# Autodesk Inventor assembly: robotic_guitar
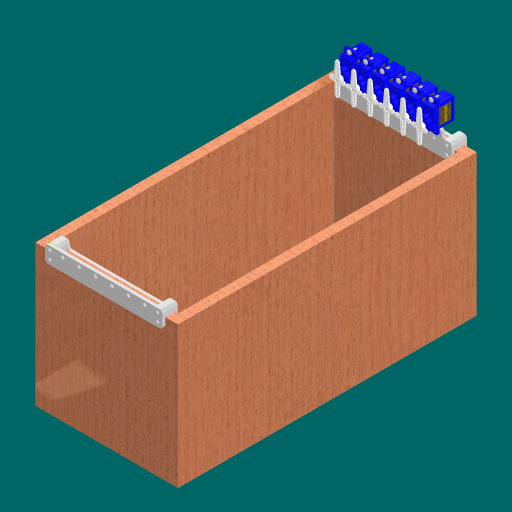
[picture p0: Inventor's stored thumbnail of the model, 512x512]
Saved by Autodesk Inventor 2023 (Build 270158000, 158)
## iProperties
Created: 2022-11-12
Part Number: robotic_guitar
Document SubType Name: Assembly
Designer: sgodi
Author: sgodi
## Documents named in this file (6)
- C:\Users\sgodi\OneDrive\Documents\CPSC 334\CPSC_334\Project4\Task 2\cad_files\robotic_guitar.iam
- C:\Users\sgodi\OneDrive\Documents\Sound Box.ipt
- C:\Users\sgodi\OneDrive\Documents\CPSC 334\CPSC_334\Project4\Task 2\cad_files\sg90-micro-servo-9g-tower-pro-1.snapshot.3\SG90 - Micro Servo 9g - Tower Pro.iam
- C:\Users\sgodi\OneDrive\Documents\CPSC 334\CPSC_334\Project4\Task 2\cad_files\servo_mount.ipt
- C:\Users\sgodi\OneDrive\Documents\CPSC 334\CPSC_334\Project4\Task 2\cad_files\servo_mount_2.ipt
- C:\Users\sgodi\OneDrive\Documents\CPSC 334\CPSC_334\Project4\Task 2\cad_files\string_mount.ipt
## Components (11 placed, 6 different names)
1. Sound Box:1 — Mate:3, Mate:4
2. SG90 - Micro Servo 9g - Tower Pro:1 [sub-assembly] — Flush:3, Flush:4, Flush:10, Tangent:6
3. SG90 - Micro Servo 9g - Tower Pro:2 [sub-assembly] — Flush:1, Flush:2, Flush:3, Flush:9, Flush:10, Tangent:5
4. SG90 - Micro Servo 9g - Tower Pro:3 [sub-assembly] — Flush:1, Flush:8, Flush:9, Tangent:4
5. SG90 - Micro Servo 9g - Tower Pro:4 [sub-assembly] — Flush:2, Flush:7, Flush:8, Tangent:3
6. SG90 - Micro Servo 9g - Tower Pro:5 [sub-assembly] — Flush:4, Flush:5, Flush:6, Flush:7, Tangent:2
7. SG90 - Micro Servo 9g - Tower Pro:6 [sub-assembly] — Flush:5, Flush:6, Mate:1, Mate:2, Tangent:1
8. servo_mount_1:1 — Flush:11, Flush:12, Flush:13, Flush:14
9. servo_mount_2:1 — Flush:12, Flush:13, Mate:1, Mate:2, Tangent:1, Tangent:2, Tangent:3, Tangent:4, Tangent:5, Tangent:6
10. string_mount:1 — Flush:15
11. servo_mount:2 — Mate:3, Mate:4, Flush:14, Flush:15
## Relationships (25: Flush 15, Tangent 6, Mate 4)
- Flush:1: SG90 - Micro Servo 9g - Tower Pro:2 ↔ SG90 - Micro Servo 9g - Tower Pro:3
- Flush:2: SG90 - Micro Servo 9g - Tower Pro:2 ↔ SG90 - Micro Servo 9g - Tower Pro:4
- Flush:3: SG90 - Micro Servo 9g - Tower Pro:1 ↔ SG90 - Micro Servo 9g - Tower Pro:2
- Flush:4: SG90 - Micro Servo 9g - Tower Pro:1 ↔ SG90 - Micro Servo 9g - Tower Pro:5
- Flush:5: SG90 - Micro Servo 9g - Tower Pro:5 ↔ SG90 - Micro Servo 9g - Tower Pro:6
- Flush:6: SG90 - Micro Servo 9g - Tower Pro:5 ↔ SG90 - Micro Servo 9g - Tower Pro:6
- Flush:7: SG90 - Micro Servo 9g - Tower Pro:4 ↔ SG90 - Micro Servo 9g - Tower Pro:5
- Flush:8: SG90 - Micro Servo 9g - Tower Pro:3 ↔ SG90 - Micro Servo 9g - Tower Pro:4
- Flush:9: SG90 - Micro Servo 9g - Tower Pro:2 ↔ SG90 - Micro Servo 9g - Tower Pro:3
- Flush:10: SG90 - Micro Servo 9g - Tower Pro:1 ↔ SG90 - Micro Servo 9g - Tower Pro:2
- Flush:11: servo_mount_1:1
- Flush:12: servo_mount_1:1 ↔ servo_mount_2:1
- Flush:13: servo_mount_1:1 ↔ servo_mount_2:1
- Mate:1: SG90 - Micro Servo 9g - Tower Pro:6 ↔ servo_mount_2:1
- Mate:2: SG90 - Micro Servo 9g - Tower Pro:6 ↔ servo_mount_2:1
- Tangent:1: SG90 - Micro Servo 9g - Tower Pro:6 ↔ servo_mount_2:1
- Tangent:2: SG90 - Micro Servo 9g - Tower Pro:5 ↔ servo_mount_2:1
- Tangent:3: SG90 - Micro Servo 9g - Tower Pro:4 ↔ servo_mount_2:1
- Tangent:4: SG90 - Micro Servo 9g - Tower Pro:3 ↔ servo_mount_2:1
- Tangent:5: SG90 - Micro Servo 9g - Tower Pro:2 ↔ servo_mount_2:1
- Tangent:6: SG90 - Micro Servo 9g - Tower Pro:1 ↔ servo_mount_2:1
- Mate:3: Sound Box:1 ↔ servo_mount:2
- Mate:4: Sound Box:1 ↔ servo_mount:2
- Flush:14: servo_mount_1:1 ↔ servo_mount:2
- Flush:15: string_mount:1 ↔ servo_mount:2
